# Autodesk Inventor assembly: ASY МОО 001 отстойник осветлитель
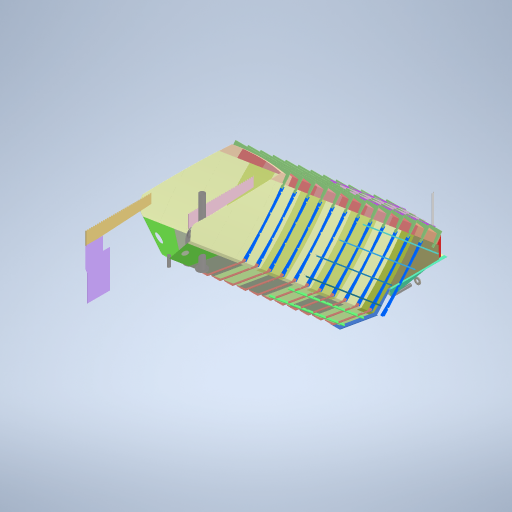
[picture p0: Inventor's stored thumbnail of the model, 512x512]
Saved by Autodesk Inventor 2024.2 (Build 282272000, 272)
## iProperties
Created: 2024-04-28
Part Number: ASY МОО 001 отстойник осветлитель
Document SubType Name: Weldment
Designer: admin
Weld Material: Welded Aluminum-6061
Mass: 1.58517e+06 g
Surface Area: 1.48953e+06 cm^2
Volume: 226523 cm^3
Density: 6.99781 g/cm^3
Author: admin
## Documents named in this file (46)
- C:\Users\admin\YandexDisk-badmisterfox\домашниий пк\Inventor\Manturovo\Manturovo_Se-clar\ASY МОО 001 отстойник осветлитель.iam
- C:\Users\admin\YandexDisk-badmisterfox\домашниий пк\Inventor\Manturovo\Manturovo_Se-clar\МОО 033 лист спина базовый.ipt
- C:\Users\admin\YandexDisk-badmisterfox\домашниий пк\Inventor\Manturovo\Manturovo_Se-clar\Пример емкости.ipt
- C:\Users\admin\YandexDisk-badmisterfox\домашниий пк\Inventor\Manturovo\Manturovo_Se-clar\МОО 041 лист брюхо основной.ipt
- C:\Users\admin\YandexDisk-badmisterfox\домашниий пк\Inventor\Manturovo\Manturovo_Se-clar\МОО 052 шпангоут борт.ipt
- C:\Users\admin\YandexDisk-badmisterfox\домашниий пк\Inventor\Manturovo\Manturovo_Se-clar\МОО 051 шпангоут спина.ipt
- C:\Users\admin\YandexDisk-badmisterfox\домашниий пк\Inventor\Manturovo\Manturovo_Se-clar\Рама основания\ASY МОО 040 рама основания.iam
- C:\Users\admin\YandexDisk-badmisterfox\домашниий пк\Inventor\Manturovo\Manturovo_Se-clar\ASY МОО 060 ракета.iam
- C:\Users\admin\YandexDisk-badmisterfox\домашниий пк\Inventor\Manturovo\Manturovo_Se-clar\Content Center Files\en-US\ISO 5251 B 3D\ISO 5251 Bends 3D without straight ends(90 deg) DN80 2 2.ipt
- C:\Users\admin\YandexDisk-badmisterfox\домашниий пк\Inventor\Manturovo\Manturovo_Se-clar\Content Center Files\en-US\ISO 5251(1)\ISO 5251 Concentric reducers DN80 x DN65 3,2 3,2.ipt
- C:\Users\admin\YandexDisk-badmisterfox\домашниий пк\Inventor\Manturovo\Manturovo_Se-clar\ASY МОО 010 конус.iam
- C:\Users\admin\YandexDisk-badmisterfox\домашниий пк\Inventor\Manturovo\Manturovo_Se-clar\ракета\МОО 064 ракета труба.ipt
- C:\Users\admin\YandexDisk-badmisterfox\домашниий пк\Inventor\Manturovo\Manturovo_Se-clar\х_размеры МОО отстойник осветлитель Dummu.ipt
- C:\Users\admin\YandexDisk-badmisterfox\домашниий пк\Inventor\Manturovo\Manturovo_Se-clar\МОО 031 лист спина поясница.ipt
- C:\Users\admin\YandexDisk-badmisterfox\домашниий пк\Inventor\Manturovo\Manturovo_Se-clar\Content Center Files\en-US\DIN EN 1092-1 01 - PN 25\DIN EN 1092-1 Plate Flange for Welding Type 01 - PN 25 80 x 88.9.ipt
- C:\Users\admin\YandexDisk-badmisterfox\домашниий пк\Inventor\Manturovo\Manturovo_Se-clar\МОО 024 лист борт основной.ipt
- C:\Users\admin\YandexDisk-badmisterfox\домашниий пк\Inventor\Manturovo\Manturovo_Se-clar\МОО 032 лист спина-поясница магич.ipt
- C:\Users\admin\YandexDisk-badmisterfox\домашниий пк\Inventor\Manturovo\Manturovo_Se-clar\МОО 021 лист левый борт бедро.ipt
- C:\Users\admin\YandexDisk-badmisterfox\домашниий пк\Inventor\Manturovo\Manturovo_Se-clar\МОО 022 лист правый борт бедро.ipt
- C:\Users\admin\YandexDisk-badmisterfox\домашниий пк\Inventor\Manturovo\Manturovo_Se-clar\МОО 034 лист спина-холка.ipt
- C:\Users\admin\YandexDisk-badmisterfox\домашниий пк\Inventor\Manturovo\Manturovo_Se-clar\МОО 042 лист брюхо-горло.ipt
- C:\Users\admin\YandexDisk-badmisterfox\домашниий пк\Inventor\Manturovo\Manturovo_Se-clar\МОО 023 лист борт.ipt
- C:\Users\admin\YandexDisk-badmisterfox\домашниий пк\Inventor\Manturovo\Manturovo_Se-clar\конус\МОО 071 гребень 1.ipt
- C:\Users\admin\YandexDisk-badmisterfox\домашниий пк\Inventor\Manturovo\Manturovo_Se-clar\конус\МОО 072 гребень 2.ipt
- C:\Users\admin\YandexDisk-badmisterfox\домашниий пк\Inventor\Manturovo\Manturovo_Se-clar\конус\МОО 073 морда 3.ipt
- C:\Users\admin\YandexDisk-badmisterfox\домашниий пк\Inventor\Manturovo\Manturovo_Se-clar\Content Center Files\en-US\ISO 5251 B 3D\ISO 5251 Bends 3D without straight ends(90 deg) DN150 11 11.ipt
- C:\Users\admin\YandexDisk-badmisterfox\домашниий пк\Inventor\Manturovo\Manturovo_Se-clar\Content Center Files\en-US\DIN EN 1092-1 01 - PN 25\DIN EN 1092-1 Plate Flange for Welding Type 01 - PN 25 150 x 168.3.ipt
- C:\Users\admin\YandexDisk-badmisterfox\домашниий пк\Inventor\Manturovo\Manturovo_Se-clar\МОО 061 труба верх 1.ipt
- C:\Users\admin\YandexDisk-badmisterfox\домашниий пк\Inventor\Manturovo\Manturovo_Se-clar\МОО 062 труба верх 2.ipt
- C:\Users\admin\YandexDisk-badmisterfox\домашниий пк\Inventor\Manturovo\Manturovo_Se-clar\МОО 063 труба верх 3.ipt
- C:\Users\admin\YandexDisk-badmisterfox\домашниий пк\Inventor\Manturovo\Manturovo_Se-clar\МОО 061 стрингер спина ^.ipt
- C:\Users\admin\YandexDisk-badmisterfox\домашниий пк\Inventor\Manturovo\Manturovo_Se-clar\МОО 063 стрингер борт #.ipt
- C:\Users\admin\YandexDisk-badmisterfox\домашниий пк\Inventor\Manturovo\Manturovo_Se-clar\МОО 062 стрингер спина ^^.ipt
- C:\Users\admin\YandexDisk-badmisterfox\домашниий пк\Inventor\Manturovo\Manturovo_Se-clar\МОО 064 стрингер борт ##.ipt
- C:\Users\admin\YandexDisk-badmisterfox\домашниий пк\Inventor\Manturovo\Manturovo_Se-clar\МОО 065 стрингер борт ###.ipt
- C:\Users\admin\YandexDisk-badmisterfox\домашниий пк\Inventor\Manturovo\Manturovo_Se-clar\МОО 066 стрингер борт ####.ipt
- C:\Users\admin\YandexDisk-badmisterfox\домашниий пк\Inventor\Manturovo\Manturovo_Se-clar\МОО 067 стрингер борт живот.ipt
- C:\Users\admin\YandexDisk-badmisterfox\домашниий пк\Inventor\Manturovo\Manturovo_Se-clar\МОО 053 шпангоут брюхо.ipt
- C:\Users\admin\YandexDisk-badmisterfox\домашниий пк\Inventor\Manturovo\Manturovo_Se-clar\МОО 025 лист борт холка.ipt
- C:\Users\admin\YandexDisk-badmisterfox\домашниий пк\Inventor\Manturovo\Manturovo_Se-clar\МОО 026 лист борт морда.ipt
- C:\Users\admin\YandexDisk-badmisterfox\домашниий пк\Inventor\Manturovo\Manturovo_Se-clar\Part1.ipt
- C:\Users\admin\YandexDisk-badmisterfox\домашниий пк\Inventor\Manturovo\Manturovo_Se-clar\стапель\ASY стапель.iam
- C:\Users\admin\YandexDisk-badmisterfox\домашниий пк\Inventor\Manturovo\Manturovo_Se-clar\DXF файлы\Шпангоуты+стрингеры\МОО 0100.ipt
- C:\Users\admin\YandexDisk-badmisterfox\домашниий пк\Inventor\Manturovo\Manturovo_Se-clar\МОО 025 лист борт холка_MIR.ipt
- C:\Users\admin\YandexDisk-badmisterfox\домашниий пк\Inventor\Manturovo\Manturovo_Se-clar\МОО 026 лист борт морда_MIR.ipt
- C:\Users\admin\YandexDisk-badmisterfox\домашниий пк\Inventor\Manturovo\Manturovo_Se-clar\МОО 068 stringer lowerback.ipt
## Components (162 placed, 55 different names)
1. Пример емкости.ipt:1 — Mate:1, Mate:2, Flush:2
2. х_размеры МОО отстойник осветлитель Dummu.ipt:1
3. ASY МОО 040 рама основания.iam:1 [sub-assembly] — Flush:19, Flush:20, Flush:21
4. МОО 033 лист спина базовый.ipt:1 — Flush:3, Rigid:11, Rigid:12
5. МОО 041 лист брюхо основной.ipt:1 — Mate:9, Rigid:18, Rigid:40
6. ASY МОО 060 ракета.iam:1 [sub-assembly] — Flush:23, Rigid:10
7. ISO 5251 Bends 3D without straight ends(90 deg) DN80 2 2.ipt:1 — Rigid:2, Rigid:3
8. ISO 5251 Concentric reducers DN80 x DN65 3,2 3,2.ipt:1 — Rigid:2, Rigid:10
9. ASY МОО 010 конус.iam:1 [sub-assembly] — Flush:22, Mate:16, Flush:28, Mate:31, Mate:36, Mate:54, Mate:57, Mate:65
10. МОО 064 ракета труба.ipt:1 — Rigid:3, Cylindrical:1
11. МОО 033 лист спина базовый.ipt:2 — Rigid:11, Tangent:1, Tangent:3, Rigid:37
12. МОО 033 лист спина базовый.ipt:3 — Flush:24, Rigid:12, Mate:19, Mate:22, Rigid:30, Mate:31, Flush:44, Tangent:8, Tangent:9
13. МОО 031 лист спина поясница.ipt:1 — Mate:15, Mate:16, Flush:27, Mate:19, Mate:22, Tangent:10
14. DIN EN 1092-1 Plate Flange for Welding Type 01 - PN 25 80 x 88.9.ipt:1 — Flush:25, Flush:26, Mate:18, Cylindrical:1
15. МОО 024 лист борт основной.ipt:1 — Flush:30, Tangent:1, Rigid:35, Mate:37
16. МОО 041 лист брюхо основной.ipt:2 — Rigid:18, Rigid:53
17. МОО 032 лист спина-поясница магич.ipt:1 — Mate:24, Rigid:30, Flush:42, Tangent:6, Flush:43, Tangent:7
18. МОО 021 лист левый борт бедро.ipt:1 — Flush:41, Flush:42, Tangent:6
19. МОО 022 лист правый борт бедро.ipt:1 — Mate:30, Flush:43, Tangent:7
20. МОО 024 лист борт основной.ipt:2 — Rigid:35, Rigid:36
21. МОО 024 лист борт основной.ipt:3 — Rigid:36, Rigid:49
22. МОО 033 лист спина базовый.ipt:4 — Rigid:37, Rigid:38
23. МОО 033 лист спина базовый.ipt:5 — Rigid:38, Rigid:39
24. МОО 034 лист спина-холка.ipt:1 — Rigid:39
25. МОО 041 лист брюхо основной.ipt:3 — Rigid:40, Rigid:47
26. МОО 042 лист брюхо-горло.ipt:1 — Rigid:48, Mate:52, Mate:53, Rigid:54
27. МОО 041 лист брюхо основной.ipt:4 — Rigid:45, Rigid:47
28. МОО 041 лист брюхо основной.ipt:5 — Rigid:45, Rigid:48
29. МОО 024 лист борт основной.ipt:4 — Rigid:49, Rigid:50
30. МОО 024 лист борт основной.ipt:5 — Rigid:50, Rigid:113
31. МОО 023 лист борт.ipt:1 — Mate:36, Flush:47, Tangent:8, Mate:37, Mate:55
32. МОО 071 гребень 1.ipt:1 — Mate:50, Flush:48
33. МОО 072 гребень 2.ipt:1
34. МОО 073 морда 3.ipt:1 — Mate:51, Mate:52, Rigid:52, Mate:53, Mate:59, Flush:49
35. МОО 073 морда 3.ipt:2 — Rigid:52, Flush:48
36. МОО 041 лист брюхо основной.ipt:6 — Mate:54, Mate:55, Rigid:53
37. DIN EN 1092-1 Plate Flange for Welding Type 01 - PN 25 80 x 88.9.ipt:2 — Rigid:54, Rigid:62
38. МОО 071 гребень 1.ipt:2
39. МОО 072 гребень 2.ipt:2 — Mate:59, Flush:49
40. DIN EN 1092-1 Plate Flange for Welding Type 01 - PN 25 150 x 168.3.ipt:1 — Rotational:1
41. МОО 061 труба верх 1.ipt:1 — Rotational:1, Rigid:59
42. ISO 5251 Bends 3D without straight ends(90 deg) DN150 11 11.ipt:1 — Rigid:59
43. МОО 062 труба верх 2.ipt:1 — Rigid:132
44. DIN EN 1092-1 Plate Flange for Welding Type 01 - PN 25 150 x 168.3.ipt:2 — Rigid:132
45. МОО 063 труба верх 3.ipt:1 — Rigid:62
46. МОО 024 лист борт основной.ipt:6 — Rigid:134
47. МОО 024 лист борт основной.ipt:7
48. МОО 024 лист борт основной.ipt:8
49. МОО 024 лист борт основной.ipt:9
50. МОО 024 лист борт основной.ipt:10 — Rigid:67
51. МОО 023 лист борт.ipt:2 — Rigid:67, Mate:57, Mate:58, Tangent:9
52. МОО 052 шпангоут борт.ipt:1 — Rigid:74, Rigid:128, Rigid:129
53. МОО 051 шпангоут спина.ipt:1 — Rigid:25, Rigid:74, Rigid:91, Rigid:93, Rigid:139
54. МОО 066 стрингер борт ####.ipt:1 — Rigid:143
55. МОО 065 стрингер борт ###.ipt:1 — Rigid:142
56. МОО 064 стрингер борт ##.ipt:1 — Rigid:129, Rigid:141
57. МОО 063 стрингер борт #.ipt:1 — Rigid:128, Rigid:140
58. МОО 062 стрингер спина ^^.ipt:1 — Rigid:93, Rigid:155
59. МОО 061 стрингер спина ^.ipt:2 — Rigid:91, Rigid:153
60. МОО 061 стрингер спина ^.ipt:1 — Rigid:90, Rigid:152
61. МОО 025 лист борт холка.ipt:1 — Rigid:113, Rigid:114
62. МОО 026 лист борт морда.ipt:1 — Rigid:114
63. Part1.ipt:1
64. МОО 051 шпангоут спина.ipt:2 — Rigid:116, Rigid:121, Rigid:130, Rigid:131
65. МОО 051 шпангоут спина.ipt:3 — Rigid:116
66. МОО 051 шпангоут спина.ipt:4 — Rigid:131
67. МОО 051 шпангоут спина.ipt:5 — Mate:62, Flush:53
68. МОО 052 шпангоут борт.ipt:2 — Rigid:121
69. МОО 062 стрингер спина ^^.ipt:2 — Rigid:92, Mate:66, Rigid:154
70. МОО 066 стрингер борт ####.ipt:2 — Rigid:125, Rigid:151
71. МОО 063 стрингер борт #.ipt:2 — Rigid:122, Rigid:148
72. МОО 064 стрингер борт ##.ipt:2 — Rigid:123, Rigid:149
73. МОО 065 стрингер борт ###.ipt:2 — Rigid:124, Rigid:150
74. МОО 052 шпангоут борт.ipt:3 — Rigid:72, Rigid:122, Rigid:123, Flush:51, Flush:52, Rigid:124, Rigid:125, Mate:61
75. МОО 051 шпангоут спина.ipt:6 — Flush:12, Tangent:3, Rigid:25, Flush:44, Rigid:72, Rigid:90, Rigid:92, Rigid:130
76. ASY стапель.iam:1 [sub-assembly] — Mate:62, Flush:53, Mate:63
77. МОО 053 шпангоут брюхо.ipt:2 — Rigid:110, Flush:51, Flush:52, Rigid:126, Mate:61, Rigid:127
78. МОО 053 шпангоут брюхо.ipt:1 — Rigid:111, Rigid:112, Rigid:127
79. МОО 067 стрингер борт живот.ipt:4 — Rigid:126, Rigid:147
80. МОО 067 стрингер борт живот.ipt:3 — Rigid:110, Rigid:146
81. МОО 067 стрингер борт живот.ipt:2 — Rigid:112, Rigid:144
82. МОО 067 стрингер борт живот.ipt:1 — Rigid:111, Rigid:145
83. МОО 0100.ipt:1 — Mate:64
84. МОО 025 лист борт холка_MIR:1 — Rigid:133, Rigid:134
85. МОО 026 лист борт морда_MIR:1 — Rigid:133
86. МОО 068 stringer lowerback:1 — Mate:65, Mate:66, Tangent:10
87. МОО 053 стрингер борт 3:3 — Rigid:140
88. МОО 054 стрингер борт 4:3 — Rigid:141
89. МОО 055 стрингер борт 5:3 — Rigid:142
90. МОО 056 стрингер борт 6:3 — Rigid:143
91. МОО 057 стрингер борт 7:5 — Rigid:147
92. МОО 057 стрингер борт 7:6 — Rigid:146
93. МОО 057 стрингер борт 7:9 — Rigid:144
94. МОО 057 стрингер борт 7:10 — Rigid:145
95. МОО 053 стрингер борт 3:4 — Rigid:148
96. МОО 054 стрингер борт 4:4 — Rigid:149
97. МОО 055 стрингер борт 5:4 — Rigid:150
98. МОО 056 стрингер борт 6:4 — Rigid:151
99. МОО 051 стрингер спина 1:3 — Rigid:153
100. МОО 051 стрингер спина 1:4 — Rigid:152
101. МОО 052 стрингер спина 2:3 — Rigid:155
102. МОО 052 стрингер спина 2:4 — Rigid:154
103. МОО 042 шпангоут брюхо:4
104. МОО 052 шпангоут борт:5
105. МОО 051 шпангоут спина:31 — Rigid:139
106. МОО 051 шпангоут спина:30
107. МОО 052 шпангоут борт:4
108. МОО 042 шпангоут брюхо:3
109. МОО 042 шпангоут брюхо:5
110. МОО 052 шпангоут борт:6
111. МОО 051 шпангоут спина:32
112. МОО 051 шпангоут спина:33
113. МОО 052 шпангоут борт:7
114. МОО 042 шпангоут брюхо:6
115. МОО 042 шпангоут брюхо:7
116. МОО 052 шпангоут борт:8
117. МОО 051 шпангоут спина:34
118. МОО 051 шпангоут спина:35
119. МОО 052 шпангоут борт:9
120. МОО 042 шпангоут брюхо:8
121. МОО 042 шпангоут брюхо:9
122. МОО 052 шпангоут борт:10
123. МОО 051 шпангоут спина:36
124. МОО 051 шпангоут спина:37
125. МОО 052 шпангоут борт:11
126. МОО 042 шпангоут брюхо:10
127. МОО 042 шпангоут брюхо:11
128. МОО 052 шпангоут борт:12
129. МОО 051 шпангоут спина:38
130. МОО 051 шпангоут спина:39
131. МОО 052 шпангоут борт:13
132. МОО 042 шпангоут брюхо:12
133. МОО 042 шпангоут брюхо:13
134. МОО 052 шпангоут борт:14
135. МОО 051 шпангоут спина:40
136. МОО 051 шпангоут спина:41
137. МОО 052 шпангоут борт:15
138. МОО 042 шпангоут брюхо:14
139. МОО 042 шпангоут брюхо:15
140. МОО 052 шпангоут борт:16
141. МОО 051 шпангоут спина:42
142. МОО 051 шпангоут спина:43
143. МОО 052 шпангоут борт:17
144. МОО 042 шпангоут брюхо:16
145. МОО 042 шпангоут брюхо:17
146. МОО 052 шпангоут борт:18
147. МОО 051 шпангоут спина:44
148. МОО 051 шпангоут спина:45
149. МОО 052 шпангоут борт:19
150. МОО 042 шпангоут брюхо:18
151. МОО 042 шпангоут брюхо:19
152. МОО 052 шпангоут борт:20
153. МОО 051 шпангоут спина:46
154. МОО 051 шпангоут спина:47
155. МОО 052 шпангоут борт:21
156. МОО 042 шпангоут брюхо:20
157. МОО 042 шпангоут брюхо:21
158. МОО 052 шпангоут борт:22
159. МОО 051 шпангоут спина:48
160. МОО 051 шпангоут спина:49
161. МОО 052 шпангоут борт:23
162. МОО 042 шпангоут брюхо:22
## Component patterns: (10 elements, first: МОО 042 шпангоут брюхо:4 + МОО 052 шпангоут борт:5 + МОО 051 шпангоут спина:31 + МОО 051 шпангоут спина:30 + МОО 052 шпангоут борт:4 + МОО 042 шпангоут брюхо:3)
## Relationships (141: WeldJoint 77, Mate 29, Flush 26, Tangent 7, CylindricalJoint 1, RevoluteJoint 1)
- Mate:1: Пример емкости.ipt:1
- Mate:2: Пример емкости.ipt:1
- Flush:2: Пример емкости.ipt:1
- Flush:3: МОО 033 лист спина базовый.ipt:1
- Mate:9: МОО 041 лист брюхо основной.ipt:1
- Flush:12: МОО 051 шпангоут спина.ipt:6
- Rigid:2 [WeldJoint]: ISO 5251 Bends 3D without straight ends(90 deg) DN80 2 2.ipt:1 ↔ ISO 5251 Concentric reducers DN80 x DN65 3,2 3,2.ipt:1
- Rigid:3 [WeldJoint]: ISO 5251 Bends 3D without straight ends(90 deg) DN80 2 2.ipt:1 ↔ МОО 064 ракета труба.ipt:1
- Flush:19 (-250 mm): ASY МОО 040 рама основания.iam:1
- Flush:20: ASY МОО 040 рама основания.iam:1
- Flush:21: ASY МОО 040 рама основания.iam:1
- Flush:22: ASY МОО 010 конус.iam:1
- Flush:23: ASY МОО 060 ракета.iam:1
- Mate:15: МОО 031 лист спина поясница.ipt:1
- Flush:24: МОО 033 лист спина базовый.ipt:3
- Mate:16: ASY МОО 010 конус.iam:1 ↔ МОО 031 лист спина поясница.ipt:1
- Flush:25: DIN EN 1092-1 Plate Flange for Welding Type 01 - PN 25 80 x 88.9.ipt:1
- Flush:26: DIN EN 1092-1 Plate Flange for Welding Type 01 - PN 25 80 x 88.9.ipt:1
- Mate:18 (120 mm): DIN EN 1092-1 Plate Flange for Welding Type 01 - PN 25 80 x 88.9.ipt:1
- Rigid:10 [WeldJoint] (-20 mm): ASY МОО 060 ракета.iam:1 ↔ ISO 5251 Concentric reducers DN80 x DN65 3,2 3,2.ipt:1
- Cylindrical:1: МОО 064 ракета труба.ipt:1 ↔ DIN EN 1092-1 Plate Flange for Welding Type 01 - PN 25 80 x 88.9.ipt:1
- Flush:27 (15 mm): МОО 031 лист спина поясница.ipt:1
- Flush:28: ASY МОО 010 конус.iam:1
- Rigid:11 [WeldJoint]: МОО 033 лист спина базовый.ipt:1 ↔ МОО 033 лист спина базовый.ipt:2
- Rigid:12 [WeldJoint]: МОО 033 лист спина базовый.ipt:1 ↔ МОО 033 лист спина базовый.ipt:3
- Mate:19 (910 mm): МОО 033 лист спина базовый.ipt:3 ↔ МОО 031 лист спина поясница.ipt:1
- Flush:30: МОО 024 лист борт основной.ipt:1
- Tangent:1: МОО 033 лист спина базовый.ipt:2 ↔ МОО 024 лист борт основной.ipt:1
- Tangent:3: МОО 033 лист спина базовый.ipt:2 ↔ МОО 051 шпангоут спина.ipt:6
- Mate:22 (47 mm): МОО 033 лист спина базовый.ipt:3 ↔ МОО 031 лист спина поясница.ipt:1
- Rigid:18 [WeldJoint]: МОО 041 лист брюхо основной.ipt:1 ↔ МОО 041 лист брюхо основной.ipt:2
- Rigid:25 [WeldJoint] (-50 mm): МОО 051 шпангоут спина.ipt:1 ↔ МОО 051 шпангоут спина.ipt:6
- Mate:24: МОО 032 лист спина-поясница магич.ipt:1
- Rigid:30 [WeldJoint]: МОО 033 лист спина базовый.ipt:3 ↔ МОО 032 лист спина-поясница магич.ipt:1
- Flush:41: МОО 021 лист левый борт бедро.ipt:1
- Flush:42: МОО 032 лист спина-поясница магич.ipt:1 ↔ МОО 021 лист левый борт бедро.ipt:1
- Tangent:6: МОО 032 лист спина-поясница магич.ipt:1 ↔ МОО 021 лист левый борт бедро.ipt:1
- Mate:30: МОО 022 лист правый борт бедро.ipt:1
- Flush:43: МОО 032 лист спина-поясница магич.ipt:1 ↔ МОО 022 лист правый борт бедро.ipt:1
- Tangent:7: МОО 032 лист спина-поясница магич.ipt:1 ↔ МОО 022 лист правый борт бедро.ipt:1
- Rigid:35 [WeldJoint]: МОО 024 лист борт основной.ipt:1 ↔ МОО 024 лист борт основной.ipt:2
- Rigid:36 [WeldJoint]: МОО 024 лист борт основной.ipt:2 ↔ МОО 024 лист борт основной.ipt:3
- Rigid:37 [WeldJoint]: МОО 033 лист спина базовый.ipt:2 ↔ МОО 033 лист спина базовый.ipt:4
- Rigid:38 [WeldJoint]: МОО 033 лист спина базовый.ipt:4 ↔ МОО 033 лист спина базовый.ipt:5
- Rigid:39 [WeldJoint]: МОО 033 лист спина базовый.ipt:5 ↔ МОО 034 лист спина-холка.ipt:1
- Mate:31: ASY МОО 010 конус.iam:1 ↔ МОО 033 лист спина базовый.ipt:3
- Rigid:40 [WeldJoint]: МОО 041 лист брюхо основной.ipt:1 ↔ МОО 041 лист брюхо основной.ipt:3
- Flush:44 (-250 mm): МОО 033 лист спина базовый.ipt:3 ↔ МОО 051 шпангоут спина.ipt:6
- Rigid:45 [WeldJoint]: МОО 041 лист брюхо основной.ipt:4 ↔ МОО 041 лист брюхо основной.ipt:5
- Rigid:47 [WeldJoint]: МОО 041 лист брюхо основной.ipt:3 ↔ МОО 041 лист брюхо основной.ipt:4
- Rigid:48 [WeldJoint]: МОО 042 лист брюхо-горло.ipt:1 ↔ МОО 041 лист брюхо основной.ipt:5
- Rigid:49 [WeldJoint]: МОО 024 лист борт основной.ipt:3 ↔ МОО 024 лист борт основной.ipt:4
- Rigid:50 [WeldJoint]: МОО 024 лист борт основной.ipt:4 ↔ МОО 024 лист борт основной.ipt:5
- Mate:36: ASY МОО 010 конус.iam:1 ↔ МОО 023 лист борт.ipt:1
- Flush:47: МОО 023 лист борт.ipt:1
- Tangent:8: МОО 033 лист спина базовый.ipt:3 ↔ МОО 023 лист борт.ipt:1
- Mate:37: МОО 024 лист борт основной.ipt:1 ↔ МОО 023 лист борт.ipt:1
- Mate:50 (200 mm): МОО 071 гребень 1.ipt:1
- Mate:51: МОО 073 морда 3.ipt:1
- Mate:52: МОО 042 лист брюхо-горло.ipt:1 ↔ МОО 073 морда 3.ipt:1
- Rigid:52 [WeldJoint]: МОО 073 морда 3.ipt:1 ↔ МОО 073 морда 3.ipt:2
- Mate:53 (-10 mm): МОО 042 лист брюхо-горло.ipt:1 ↔ МОО 073 морда 3.ipt:1
- Mate:54: ASY МОО 010 конус.iam:1 ↔ МОО 041 лист брюхо основной.ipt:6
- Mate:55: МОО 023 лист борт.ipt:1 ↔ МОО 041 лист брюхо основной.ipt:6
- Rigid:53 [WeldJoint]: МОО 041 лист брюхо основной.ipt:2 ↔ МОО 041 лист брюхо основной.ipt:6
- Rigid:54 [WeldJoint] (200 mm): МОО 042 лист брюхо-горло.ipt:1 ↔ DIN EN 1092-1 Plate Flange for Welding Type 01 - PN 25 80 x 88.9.ipt:2
- Flush:48 (-200 mm): МОО 071 гребень 1.ipt:1 ↔ МОО 073 морда 3.ipt:2
- Rotational:1 [RevoluteJoint]: DIN EN 1092-1 Plate Flange for Welding Type 01 - PN 25 150 x 168.3.ipt:1 ↔ МОО 061 труба верх 1.ipt:1
- Rigid:59 [WeldJoint]: МОО 061 труба верх 1.ipt:1 ↔ ISO 5251 Bends 3D without straight ends(90 deg) DN150 11 11.ipt:1
- Rigid:62 [WeldJoint]: DIN EN 1092-1 Plate Flange for Welding Type 01 - PN 25 80 x 88.9.ipt:2 ↔ МОО 063 труба верх 3.ipt:1
- [WeldJoint]: МОО 024 лист борт основной.ipt:6 ↔ МОО 024 лист борт основной.ipt:7
- [WeldJoint]: МОО 024 лист борт основной.ipt:7 ↔ МОО 024 лист борт основной.ipt:8
- [WeldJoint]: МОО 024 лист борт основной.ipt:8 ↔ МОО 024 лист борт основной.ipt:9
- [WeldJoint]: МОО 024 лист борт основной.ipt:9 ↔ МОО 024 лист борт основной.ipt:10
- Rigid:67 [WeldJoint]: МОО 024 лист борт основной.ipt:10 ↔ МОО 023 лист борт.ipt:2
- Mate:57: ASY МОО 010 конус.iam:1 ↔ МОО 023 лист борт.ipt:2
- Mate:58: МОО 023 лист борт.ipt:2
- Tangent:9: МОО 033 лист спина базовый.ipt:3 ↔ МОО 023 лист борт.ipt:2
- Rigid:72 [WeldJoint] (-50 mm): МОО 052 шпангоут борт.ipt:3 ↔ МОО 051 шпангоут спина.ipt:6
- Rigid:74 [WeldJoint] (-50 mm): МОО 052 шпангоут борт.ipt:1 ↔ МОО 051 шпангоут спина.ipt:1
- Rigid:90 [WeldJoint] (2 mm): МОО 061 стрингер спина ^.ipt:1 ↔ МОО 051 шпангоут спина.ipt:6
- Rigid:91 [WeldJoint] (2 mm): МОО 051 шпангоут спина.ipt:1 ↔ МОО 061 стрингер спина ^.ipt:2
- Rigid:92 [WeldJoint] (2 mm): МОО 062 стрингер спина ^^.ipt:2 ↔ МОО 051 шпангоут спина.ipt:6
- Rigid:93 [WeldJoint] (2 mm): МОО 051 шпангоут спина.ipt:1 ↔ МОО 062 стрингер спина ^^.ipt:1
- Rigid:110 [WeldJoint] (2 mm): МОО 053 шпангоут брюхо.ipt:2 ↔ МОО 067 стрингер борт живот.ipt:3
- Rigid:111 [WeldJoint] (2 mm): МОО 053 шпангоут брюхо.ipt:1 ↔ МОО 067 стрингер борт живот.ipt:1
- Rigid:112 [WeldJoint] (2 mm): МОО 053 шпангоут брюхо.ipt:1 ↔ МОО 067 стрингер борт живот.ipt:2
- Rigid:113 [WeldJoint]: МОО 024 лист борт основной.ipt:5 ↔ МОО 025 лист борт холка.ipt:1
- Rigid:114 [WeldJoint]: МОО 025 лист борт холка.ipt:1 ↔ МОО 026 лист борт морда.ipt:1
- Rigid:116 [WeldJoint] (50 mm): МОО 051 шпангоут спина.ipt:2 ↔ МОО 051 шпангоут спина.ipt:3
- [WeldJoint] (50 mm): МОО 051 шпангоут спина.ipt:4 ↔ МОО 051 шпангоут спина.ipt:5
- Rigid:121 [WeldJoint] (-50 mm): МОО 051 шпангоут спина.ipt:2 ↔ МОО 052 шпангоут борт.ipt:2
- Rigid:122 [WeldJoint] (2 mm): МОО 063 стрингер борт #.ipt:2 ↔ МОО 052 шпангоут борт.ipt:3
- Rigid:123 [WeldJoint] (2 mm): МОО 064 стрингер борт ##.ipt:2 ↔ МОО 052 шпангоут борт.ipt:3
- Mate:59 (-450 mm): МОО 073 морда 3.ipt:1 ↔ МОО 072 гребень 2.ipt:2
- Flush:49: МОО 073 морда 3.ipt:1 ↔ МОО 072 гребень 2.ipt:2
- Flush:51: МОО 052 шпангоут борт.ipt:3 ↔ МОО 053 шпангоут брюхо.ipt:2
- Flush:52: МОО 052 шпангоут борт.ipt:3 ↔ МОО 053 шпангоут брюхо.ipt:2
- Rigid:124 [WeldJoint] (2 mm): МОО 065 стрингер борт ###.ipt:2 ↔ МОО 052 шпангоут борт.ipt:3
- Rigid:125 [WeldJoint]: МОО 066 стрингер борт ####.ipt:2 ↔ МОО 052 шпангоут борт.ipt:3
- Rigid:126 [WeldJoint] (2 mm): МОО 053 шпангоут брюхо.ipt:2 ↔ МОО 067 стрингер борт живот.ipt:4
- Mate:61: МОО 052 шпангоут борт.ipt:3 ↔ МОО 053 шпангоут брюхо.ipt:2
- Mate:62: МОО 051 шпангоут спина.ipt:5 ↔ ASY стапель.iam:1
- Flush:53: МОО 051 шпангоут спина.ipt:5 ↔ ASY стапель.iam:1
- Mate:63: ASY стапель.iam:1
- Rigid:127 [WeldJoint] (-50 mm): МОО 053 шпангоут брюхо.ipt:2 ↔ МОО 053 шпангоут брюхо.ipt:1
- Rigid:128 [WeldJoint] (2 mm): МОО 052 шпангоут борт.ipt:1 ↔ МОО 063 стрингер борт #.ipt:1
- Rigid:129 [WeldJoint] (2 mm): МОО 052 шпангоут борт.ipt:1 ↔ МОО 064 стрингер борт ##.ipt:1
- Rigid:130 [WeldJoint] (-500 mm): МОО 051 шпангоут спина.ipt:2 ↔ МОО 051 шпангоут спина.ipt:6
- Rigid:131 [WeldJoint] (-500 mm): МОО 051 шпангоут спина.ipt:2 ↔ МОО 051 шпангоут спина.ipt:4
- Rigid:132 [WeldJoint]: МОО 062 труба верх 2.ipt:1 ↔ DIN EN 1092-1 Plate Flange for Welding Type 01 - PN 25 150 x 168.3.ipt:2
- Mate:64: МОО 0100.ipt:1
- Rigid:133 [WeldJoint]: МОО 025 лист борт холка_MIR:1 ↔ МОО 026 лист борт морда_MIR:1
- Rigid:134 [WeldJoint]: МОО 024 лист борт основной.ipt:6 ↔ МОО 025 лист борт холка_MIR:1
- Mate:65: ASY МОО 010 конус.iam:1 ↔ МОО 068 stringer lowerback:1
- Mate:66: МОО 062 стрингер спина ^^.ipt:2 ↔ МОО 068 stringer lowerback:1
- Tangent:10: МОО 031 лист спина поясница.ipt:1 ↔ МОО 068 stringer lowerback:1
- [WeldJoint] (-50 mm): МОО 051 шпангоут спина:31 ↔ МОО 051 шпангоут спина:30
- [WeldJoint] (-50 mm): МОО 051 шпангоут спина:30 ↔ МОО 052 шпангоут борт:4
- [WeldJoint] (-50 mm): МОО 052 шпангоут борт:5 ↔ МОО 051 шпангоут спина:31
- [Flush]: МОО 052 шпангоут борт:4 ↔ МОО 042 шпангоут брюхо:3
- [Flush]: МОО 052 шпангоут борт:4 ↔ МОО 042 шпангоут брюхо:3
- [Mate]: МОО 052 шпангоут борт:4 ↔ МОО 042 шпангоут брюхо:3
- [WeldJoint] (-50 mm): МОО 042 шпангоут брюхо:4 ↔ МОО 042 шпангоут брюхо:3
- Rigid:139 [WeldJoint] (-500 mm): МОО 051 шпангоут спина.ipt:1 ↔ МОО 051 шпангоут спина:31
- Rigid:140 [WeldJoint]: МОО 063 стрингер борт #.ipt:1 ↔ МОО 053 стрингер борт 3:3
- Rigid:141 [WeldJoint]: МОО 064 стрингер борт ##.ipt:1 ↔ МОО 054 стрингер борт 4:3
- Rigid:142 [WeldJoint]: МОО 065 стрингер борт ###.ipt:1 ↔ МОО 055 стрингер борт 5:3
- Rigid:143 [WeldJoint]: МОО 066 стрингер борт ####.ipt:1 ↔ МОО 056 стрингер борт 6:3
- Rigid:144 [WeldJoint]: МОО 067 стрингер борт живот.ipt:2 ↔ МОО 057 стрингер борт 7:9
- Rigid:145 [WeldJoint]: МОО 067 стрингер борт живот.ipt:1 ↔ МОО 057 стрингер борт 7:10
- Rigid:146 [WeldJoint]: МОО 067 стрингер борт живот.ipt:3 ↔ МОО 057 стрингер борт 7:6
- Rigid:147 [WeldJoint]: МОО 067 стрингер борт живот.ipt:4 ↔ МОО 057 стрингер борт 7:5
- Rigid:148 [WeldJoint]: МОО 063 стрингер борт #.ipt:2 ↔ МОО 053 стрингер борт 3:4
- Rigid:149 [WeldJoint]: МОО 064 стрингер борт ##.ipt:2 ↔ МОО 054 стрингер борт 4:4
- Rigid:150 [WeldJoint]: МОО 065 стрингер борт ###.ipt:2 ↔ МОО 055 стрингер борт 5:4
- Rigid:151 [WeldJoint]: МОО 066 стрингер борт ####.ipt:2 ↔ МОО 056 стрингер борт 6:4
- Rigid:152 [WeldJoint]: МОО 061 стрингер спина ^.ipt:1 ↔ МОО 051 стрингер спина 1:4
- Rigid:153 [WeldJoint]: МОО 061 стрингер спина ^.ipt:2 ↔ МОО 051 стрингер спина 1:3
- Rigid:154 [WeldJoint]: МОО 062 стрингер спина ^^.ipt:2 ↔ МОО 052 стрингер спина 2:4
- Rigid:155 [WeldJoint]: МОО 062 стрингер спина ^^.ipt:1 ↔ МОО 052 стрингер спина 2:3
## Named parameters: Бак_нахлест_фланца = 25 mm, d230_d194 = 0 mm, d231_d195 = 0 mm, d232_d160 = 0 mm, d233_d161 = 0 mm, d322_d320 = 50 mm, d384_d346 = 0 mm, d385_d359 = -50 mm, d386_d341 = 0 mm, d387_d342 = 0 mm, d388_d243 = -50 mm, d389_d246 = -50 mm, d390_d128 = -50 mm
